# Autodesk Inventor assembly: ESAMBLE_AVILA_1072720
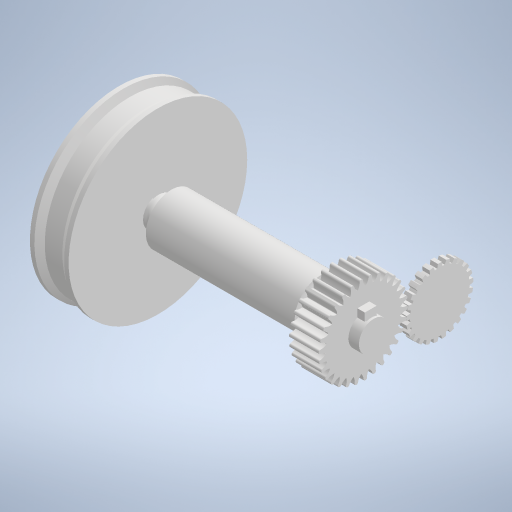
[picture p0: Inventor's stored thumbnail of the model, 512x512]
Saved by Autodesk Inventor 2024 (Build 280153000, 153)
## iProperties
Created: 2024-03-31
Part Number: ESAMBLE_AVILA_1072720
Document SubType Name: Assembly
Designer: aacas
Author: aacas
## Documents named in this file (6)
- C:\Users\aacas\Desktop\URL\Semestre No. 1\INVENTOR\ESAMBLE_AVILA_1072720.iam
- C:\Users\aacas\Downloads\EJE_CUÑEROS.ipt
- C:\Users\aacas\Downloads\POLEA.ipt
- C:\Users\aacas\Downloads\CUÑA.ipt
- C:\Users\aacas\Downloads\ENGRANE.ipt
- C:\Users\aacas\Desktop\URL\Semestre No. 1\INVENTOR\engranaje hecho por mi.ipt
## Components (6 placed, 5 different names)
1. EJE_CUÑEROS:1 — Rigid:1, Rigid:2, Mate:1, Mate:2
2. POLEA:1 — Mate:1, Flush:1
3. ENGRANE:1 — Mate:2, Mate:3, Mate:4, Flush:2
4. CUÑA:1 — Rigid:1, Flush:1
5. CUÑA:2 — Rigid:2, Mate:3
6. engranaje hecho por mi:1 — Mate:4, Flush:2
## Relationships (8: Mate 4, WeldJoint 2, Flush 2)
- Rigid:1 [WeldJoint]: EJE_CUÑEROS:1 ↔ CUÑA:1
- Rigid:2 [WeldJoint]: EJE_CUÑEROS:1 ↔ CUÑA:2
- Mate:1: EJE_CUÑEROS:1 ↔ POLEA:1
- Mate:2: EJE_CUÑEROS:1 ↔ ENGRANE:1
- Mate:3: ENGRANE:1 ↔ CUÑA:2
- Flush:1: POLEA:1 ↔ CUÑA:1
- Mate:4: ENGRANE:1 ↔ engranaje hecho por mi:1
- Flush:2: ENGRANE:1 ↔ engranaje hecho por mi:1
